# Autodesk Inventor assembly: Right Rear Wheel with hub inside_MIR
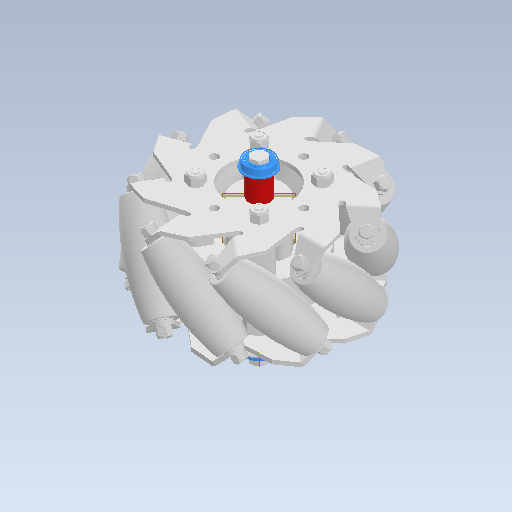
[picture p0: Inventor's stored thumbnail of the model, 512x512]
Saved by Autodesk Inventor 2020 (Build 240168000, 168)
## iProperties
Created: 2020-02-22
Part Number: Right Rear Wheel with hub inside_MIR
Document SubType Name: Assembly
Designer: jackm
Author: ball
## Documents named in this file (11)
- D:\FTC8863\2019 Robot\Mecanum Drive Train Metal\Right Rear Wheel with hub inside_MIR.iam
- D:\FTC8863\GoBilda\3213 Parts\3606-0000-0100 assembly_MIR.iam
- D:\FTC8863\StepLibraries\Screws\M4 x 22 SOCKET HEAD CAP SCREW_MIR.ipt
- D:\FTC8863\StepLibraries\Washers\M4 FLAT WASHER_MIR.ipt
- D:\FTC8863\GoBilda\1310 Parts\1310-0016-4008 assembly_MIR.ipt
- D:\FTC8863\GoBilda\2102 Parts\2102-0008-0090_MIR.ipt
- D:\FTC8863\GoBilda\3414 Parts\3414-4008-0016 assembly_MIR.iam
- D:\FTC8863\GoBilda\1601 Parts\1601-0014-0008_MIR.ipt
- D:\FTC8863\2019 Robot\Mecanum Drive Train Metal\spacer for inside of wheel_MIR.ipt
- D:\FTC8863\2019 Robot\Mecanum Drive Train Metal\spacer for outside of wheel_MIR.ipt
- D:\FTC8863\2019 Robot\Mecanum Drive Train Metal\spacer for wheel pulley_MIR.ipt
## Components (17 placed, 10 different names)
1. 3606-0000-0100 assembly_MIR:1 [sub-assembly] — Mate:31, Mate:30, Mate:29, Mate:28, Mate:27, Mate:26, Mate:43, Mate:40, Mate:46, Mate:42, Mate:45, Mate:41, Mate:54, Mate:56
2. M4 x 22 SOCKET HEAD CAP SCREW_MIR:1 — Mate:31, Mate:25, Mate:24
3. M4 FLAT WASHER_MIR:1 — Mate:30, Mate:25, Mate:24
4. 1310-0016-4008 assembly_MIR:1 — Mate:29, Mate:28, Mate:27, Mate:26, Mate:55, Mate:58
5. M4 x 22 SOCKET HEAD CAP SCREW_MIR:2 — Mate:43, Mate:33, Mate:32
6. M4 FLAT WASHER_MIR:2 — Mate:40, Mate:33, Mate:32
7. M4 x 22 SOCKET HEAD CAP SCREW_MIR:3 — Mate:46, Mate:35, Mate:34
8. M4 FLAT WASHER_MIR:3 — Mate:42, Mate:35, Mate:34
9. M4 x 22 SOCKET HEAD CAP SCREW_MIR:4 — Mate:45, Mate:37, Mate:36
10. M4 FLAT WASHER_MIR:4 — Mate:41, Mate:37, Mate:36
11. 2102-0008-0090_MIR:1 — Mate:55, Mate:54, Mate:47, Mate:48, Mate:49, Mate:53, Mate:59, Mate:61, Mate:63
12. 3414-4008-0016 assembly_MIR:1 [sub-assembly] — Mate:56, Mate:47, Mate:48, Flush:1, Mate:60, Mate:62
13. 1601-0014-0008_MIR:1 — Mate:49, Mate:64
14. 1601-0014-0008_MIR:2 — Mate:64, Flush:1, Mate:53
15. spacer for inside of wheel_MIR:1 — Mate:59, Mate:58
16. spacer for outside of wheel_MIR:1 — Mate:60, Mate:61
17. spacer for wheel pulley_MIR:1 — Mate:63, Mate:62
## Relationships (35: Mate 34, Flush 1)
- Mate:31: 3606-0000-0100 assembly_MIR:1 ↔ M4 x 22 SOCKET HEAD CAP SCREW_MIR:1
- Mate:30: 3606-0000-0100 assembly_MIR:1 ↔ M4 FLAT WASHER_MIR:1
- Mate:25: M4 x 22 SOCKET HEAD CAP SCREW_MIR:1 ↔ M4 FLAT WASHER_MIR:1
- Mate:24: M4 x 22 SOCKET HEAD CAP SCREW_MIR:1 ↔ M4 FLAT WASHER_MIR:1
- Mate:29: 3606-0000-0100 assembly_MIR:1 ↔ 1310-0016-4008 assembly_MIR:1
- Mate:28: 3606-0000-0100 assembly_MIR:1 ↔ 1310-0016-4008 assembly_MIR:1
- Mate:27: 3606-0000-0100 assembly_MIR:1 ↔ 1310-0016-4008 assembly_MIR:1
- Mate:26: 3606-0000-0100 assembly_MIR:1 ↔ 1310-0016-4008 assembly_MIR:1
- Mate:43: 3606-0000-0100 assembly_MIR:1 ↔ M4 x 22 SOCKET HEAD CAP SCREW_MIR:2
- Mate:40: 3606-0000-0100 assembly_MIR:1 ↔ M4 FLAT WASHER_MIR:2
- Mate:33: M4 x 22 SOCKET HEAD CAP SCREW_MIR:2 ↔ M4 FLAT WASHER_MIR:2
- Mate:32: M4 x 22 SOCKET HEAD CAP SCREW_MIR:2 ↔ M4 FLAT WASHER_MIR:2
- Mate:46: 3606-0000-0100 assembly_MIR:1 ↔ M4 x 22 SOCKET HEAD CAP SCREW_MIR:3
- Mate:42: 3606-0000-0100 assembly_MIR:1 ↔ M4 FLAT WASHER_MIR:3
- Mate:35: M4 x 22 SOCKET HEAD CAP SCREW_MIR:3 ↔ M4 FLAT WASHER_MIR:3
- Mate:34: M4 x 22 SOCKET HEAD CAP SCREW_MIR:3 ↔ M4 FLAT WASHER_MIR:3
- Mate:45: 3606-0000-0100 assembly_MIR:1 ↔ M4 x 22 SOCKET HEAD CAP SCREW_MIR:4
- Mate:41: 3606-0000-0100 assembly_MIR:1 ↔ M4 FLAT WASHER_MIR:4
- Mate:37: M4 x 22 SOCKET HEAD CAP SCREW_MIR:4 ↔ M4 FLAT WASHER_MIR:4
- Mate:36: M4 x 22 SOCKET HEAD CAP SCREW_MIR:4 ↔ M4 FLAT WASHER_MIR:4
- Mate:55: 1310-0016-4008 assembly_MIR:1 ↔ 2102-0008-0090_MIR:1
- Mate:54: 3606-0000-0100 assembly_MIR:1 ↔ 2102-0008-0090_MIR:1
- Mate:56 (1.27 mm): 3606-0000-0100 assembly_MIR:1 ↔ 3414-4008-0016 assembly_MIR:1
- Mate:47: 2102-0008-0090_MIR:1 ↔ 3414-4008-0016 assembly_MIR:1
- Mate:48: 2102-0008-0090_MIR:1 ↔ 3414-4008-0016 assembly_MIR:1
- Mate:49: 2102-0008-0090_MIR:1 ↔ 1601-0014-0008_MIR:1
- Mate:64 (-77.6732 mm): 1601-0014-0008_MIR:1 ↔ 1601-0014-0008_MIR:2
- Flush:1 (-3.0734 mm): 3414-4008-0016 assembly_MIR:1 ↔ 1601-0014-0008_MIR:2
- Mate:53: 2102-0008-0090_MIR:1 ↔ 1601-0014-0008_MIR:2
- Mate:59: 2102-0008-0090_MIR:1 ↔ spacer for inside of wheel_MIR:1
- Mate:58: 1310-0016-4008 assembly_MIR:1 ↔ spacer for inside of wheel_MIR:1
- Mate:60: 3414-4008-0016 assembly_MIR:1 ↔ spacer for outside of wheel_MIR:1
- Mate:61: 2102-0008-0090_MIR:1 ↔ spacer for outside of wheel_MIR:1
- Mate:63: 2102-0008-0090_MIR:1 ↔ spacer for wheel pulley_MIR:1
- Mate:62: 3414-4008-0016 assembly_MIR:1 ↔ spacer for wheel pulley_MIR:1
